# Autodesk Inventor assembly: Боковые стены
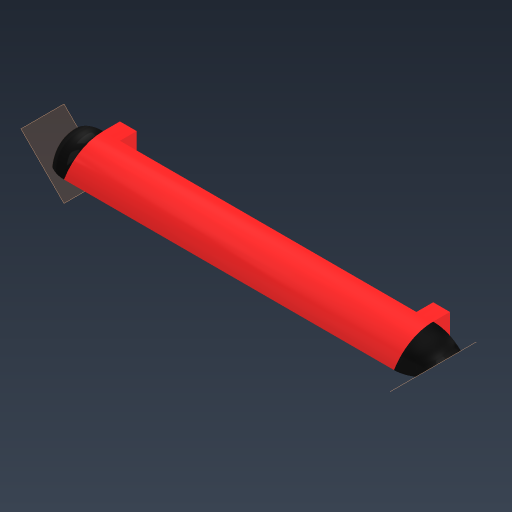
[picture p0: Inventor's stored thumbnail of the model, 512x512]
Saved by Autodesk Inventor 2023.2 (Build 272271030, 271C)
## iProperties
Created: 2025-08-19
Part Number: Боковые стены
Document SubType Name: Assembly
Designer: Олег Коноваленко
Author: Олег Коноваленко
## Documents named in this file (3)
- D:\!Rover\Rover\Rover_construction\Боковые стены.iam
- D:\!Rover\Rover\Rover_construction\Нижний край.ipt
- D:\!Rover\Rover\Rover_construction\пробник.ipt
## Components (3 placed, 2 different names)
1. Нижний край:1 — Совмещение:7, Совмещение:13, Заподлицо:3, Совмещение:16, Совмещение:17, Совмещение:18
2. пробник:1 — Совмещение:7, Совмещение:13, Заподлицо:3
3. пробник:2 — Совмещение:16, Совмещение:17, Совмещение:18
## Relationships (6: Mate 5, Flush 1)
- Совмещение:7 [Mate]: Нижний край:1 ↔ пробник:1
- Совмещение:13 [Mate]: Нижний край:1 ↔ пробник:1
- Заподлицо:3 [Flush]: Нижний край:1 ↔ пробник:1
- Совмещение:16 [Mate]: Нижний край:1 ↔ пробник:2
- Совмещение:17 [Mate]: Нижний край:1 ↔ пробник:2
- Совмещение:18 [Mate]: Нижний край:1 ↔ пробник:2
